# Autodesk Inventor assembly: AFL-102-004-01-0C RoadBot Pneumatic Module - with Jack - r4
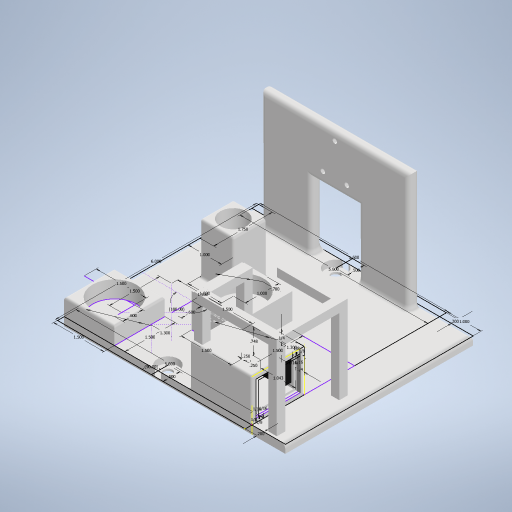
[picture p0: Inventor's stored thumbnail of the model, 512x512]
Saved by Autodesk Inventor 2024.1 (Build 281209000, 209)
## iProperties
Created: 2022-04-02
Part Number: AFL-102-004-01-0C RoadBot Pneumatic Module - with Jack - r4
Document SubType Name: Assembly
Designer: Beaucage
Author: Beaucage
## Documents named in this file (3)
- C:\Users\pab2\Documents\GitHub\AFL-hardware-devel\CAD-NewOrgScheme\AFL-102-(TravelAFL)\004-(PneumaticModule)\AFL-102-004-01-0C RoadBot Pneumatic Module - with Jack - r4.iam
- C:\Users\pab2\Documents\GitHub\AFL-hardware-devel\CAD-NewOrgScheme\AFL-102-(TravelAFL)\004-(PneumaticModule)\Keystone_Jack_Single_Receptacle (1).ipt
- C:\Users\pab2\Documents\GitHub\AFL-hardware-devel\CAD-NewOrgScheme\AFL-102-(TravelAFL)\004-(PneumaticModule)\RoadBot Pneumatic Module - Base - r4.ipt
## Components (2 placed, 2 different names)
1. RoadBot Pneumatic Module - Base - r4:1 — Mate:1, Mate:2, Flush:1
2. Keystone_Jack_Single_Receptacle (1):1 — Mate:1, Mate:2, Flush:1
## Relationships (3: Mate 2, Flush 1)
- Mate:1: RoadBot Pneumatic Module - Base - r4:1 ↔ Keystone_Jack_Single_Receptacle (1):1
- Mate:2: RoadBot Pneumatic Module - Base - r4:1 ↔ Keystone_Jack_Single_Receptacle (1):1
- Flush:1: RoadBot Pneumatic Module - Base - r4:1 ↔ Keystone_Jack_Single_Receptacle (1):1
